# Autodesk Inventor assembly: servo
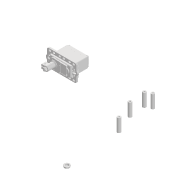
[picture p0: Inventor's stored thumbnail of the model, 180x180]
Saved by Autodesk Inventor 2020 (Build 240168000, 168)
## iProperties
Created: 2019-12-16
Part Number: servo
Document SubType Name: Assembly
Designer: ball
Author: ball
## Documents named in this file (6)
- C:\FTC\FTC8863CAD\2019 Robot\Delivery\extension arm\servo.iam
- C:\FTC\FTC8863CAD\Actobotics\575 parts\575112.ipt
- C:\FTC\FTC8863CAD\Actobotics\633 parts\633130.ipt
- C:\FTC\FTC8863CAD\Actobotics\525 parts\525150 assembly.ipt
- C:\FTC\FTC8863CAD\Actobotics\535 parts\535042.ipt
- C:\FTC\FTC8863CAD\GoBilda\2000 Parts\2000-0025-0002.ipt
## Components (8 placed, 5 different names)
1. 575112:1 — Mate:1, Mate:2, Flush:1
2. 633130:1
3. 633130:2
4. 633130:3
5. 633130:4
6. 525150 assembly:1 — Mate:3, Mate:4
7. 535042:1
8. 2000-0025-0002:1 — Mate:1, Mate:2, Flush:1, Mate:3, Mate:4
## Relationships (5: Mate 4, Flush 1)
- Mate:1: 575112:1 ↔ 2000-0025-0002:1
- Mate:2: 575112:1 ↔ 2000-0025-0002:1
- Flush:1: 575112:1 ↔ 2000-0025-0002:1
- Mate:3: 525150 assembly:1 ↔ 2000-0025-0002:1
- Mate:4: 525150 assembly:1 ↔ 2000-0025-0002:1
